# Autodesk Inventor assembly: ChassisFrame-SubAssem01
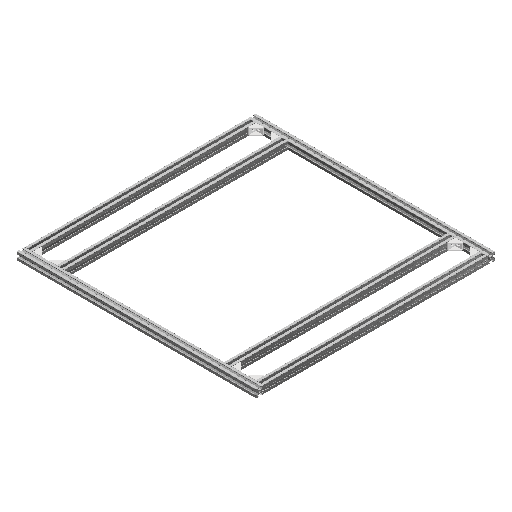
[picture p0: Inventor's stored thumbnail of the model, 512x512]
Saved by Autodesk Inventor 2024 (Build 280153000, 153)
## iProperties
Created: 2022-07-11
Part Number: ChassisFrame-SubAssem01
Document SubType Name: Assembly
Designer: Dave
Author: Dave
## Documents named in this file (5)
- C:\Autodesk\ChalkBot Github\ChalkbotMechanical\Chalkbot1.0\Chassis\V1\ChassisFrame-SubAssem01.iam
- C:\Autodesk\ChalkBot Github\ChalkbotMechanical\Chalkbot1.0\Chassis\V1\20x20 Channel\20x20 Channel-600.ipt
- C:\Users\Dave\Documents\GrabCAD\Chalk Bot\Chalkbot1.0\Chassis\20x20 Channel.ipt
- C:\Autodesk\ChalkBot Github\ChalkbotMechanical\Chalkbot1.0\Chassis\V1\20x20 Channel\20x20 Channel-560.ipt
- C:\Autodesk\ChalkBot Github\ChalkbotMechanical\Chalkbot1.0\Chassis\V1\20x20 90 Gusset.ipt
## Components (14 placed, 3 different names)
1. 20x20 Channel-600:1 — Flush:1, Flush:2, Mate:1, Flush:3, Flush:4, Flush:5, Flush:6, Flush:7, Mate:3, Flush:10, Flush:11, Flush:12, Flush:13, Mate:12, Mate:14, Mate:16, Mate:19
2. 20x20 Channel-600:2 — Flush:1, Flush:2, Mate:2, Mate:4, Mate:7, Mate:8, Mate:10
3. 20x20 Channel-560:3 — Mate:1, Flush:3, Flush:4, Mate:2, Mate:5, Mate:18, Mate:21
4. 20x20 Channel-560:4 — Flush:5, Flush:8, Mate:9, Mate:15, Mate:20
5. 20x20 Channel-560:5 — Flush:7, Flush:9, Mate:3, Flush:10, Flush:14, Flush:15, Flush:16, Flush:17, Flush:18, Mate:11, Mate:13, Mate:20
6. 20x20 Channel-560:6 — Flush:6, Flush:8, Flush:9, Mate:6, Mate:17, Mate:21
7. 20x20 90 Gusset:1 — Flush:11, Mate:12, Mate:13
8. 20x20 90 Gusset:2 — Flush:12, Mate:14, Mate:15
9. 20x20 90 Gusset:3 — Flush:13, Mate:18, Mate:19
10. 20x20 90 Gusset:4 — Flush:14, Mate:16, Mate:17
11. 20x20 90 Gusset:5 — Flush:15, Mate:8, Mate:9
12. 20x20 90 Gusset:6 — Flush:16, Mate:10, Mate:11
13. 20x20 90 Gusset:7 — Flush:17, Mate:6, Mate:7
14. 20x20 90 Gusset:8 — Flush:18, Mate:4, Mate:5
## Relationships (39: Mate 21, Flush 18)
- Flush:1: 20x20 Channel-600:1 ↔ 20x20 Channel-600:2
- Flush:2: 20x20 Channel-600:1 ↔ 20x20 Channel-600:2
- Mate:1: 20x20 Channel-600:1 ↔ 20x20 Channel-560:3
- Flush:3: 20x20 Channel-600:1 ↔ 20x20 Channel-560:3
- Flush:4: 20x20 Channel-600:1 ↔ 20x20 Channel-560:3
- Mate:2: 20x20 Channel-600:2 ↔ 20x20 Channel-560:3
- Flush:5: 20x20 Channel-600:1 ↔ 20x20 Channel-560:4
- Flush:6: 20x20 Channel-600:1 ↔ 20x20 Channel-560:6
- Flush:7: 20x20 Channel-600:1 ↔ 20x20 Channel-560:5
- Flush:8: 20x20 Channel-560:4 ↔ 20x20 Channel-560:6
- Flush:9: 20x20 Channel-560:5 ↔ 20x20 Channel-560:6
- Mate:3: 20x20 Channel-600:1 ↔ 20x20 Channel-560:5
- Flush:10: 20x20 Channel-600:1 ↔ 20x20 Channel-560:5
- Flush:11: 20x20 Channel-600:1 ↔ 20x20 90 Gusset:1
- Flush:12: 20x20 Channel-600:1 ↔ 20x20 90 Gusset:2
- Flush:13: 20x20 Channel-600:1 ↔ 20x20 90 Gusset:3
- Flush:14: 20x20 Channel-560:5 ↔ 20x20 90 Gusset:4
- Flush:15: 20x20 Channel-560:5 ↔ 20x20 90 Gusset:5
- Flush:16: 20x20 Channel-560:5 ↔ 20x20 90 Gusset:6
- Flush:17: 20x20 Channel-560:5 ↔ 20x20 90 Gusset:7
- Flush:18: 20x20 Channel-560:5 ↔ 20x20 90 Gusset:8
- Mate:4: 20x20 Channel-600:2 ↔ 20x20 90 Gusset:8
- Mate:5: 20x20 Channel-560:3 ↔ 20x20 90 Gusset:8
- Mate:6: 20x20 Channel-560:6 ↔ 20x20 90 Gusset:7
- Mate:7: 20x20 Channel-600:2 ↔ 20x20 90 Gusset:7
- Mate:8: 20x20 Channel-600:2 ↔ 20x20 90 Gusset:5
- Mate:9: 20x20 Channel-560:4 ↔ 20x20 90 Gusset:5
- Mate:10: 20x20 Channel-600:2 ↔ 20x20 90 Gusset:6
- Mate:11: 20x20 Channel-560:5 ↔ 20x20 90 Gusset:6
- Mate:12: 20x20 Channel-600:1 ↔ 20x20 90 Gusset:1
- Mate:13: 20x20 Channel-560:5 ↔ 20x20 90 Gusset:1
- Mate:14: 20x20 Channel-600:1 ↔ 20x20 90 Gusset:2
- Mate:15: 20x20 Channel-560:4 ↔ 20x20 90 Gusset:2
- Mate:16: 20x20 Channel-600:1 ↔ 20x20 90 Gusset:4
- Mate:17: 20x20 Channel-560:6 ↔ 20x20 90 Gusset:4
- Mate:18: 20x20 Channel-560:3 ↔ 20x20 90 Gusset:3
- Mate:19: 20x20 Channel-600:1 ↔ 20x20 90 Gusset:3
- Mate:20 (60 mm): 20x20 Channel-560:4 ↔ 20x20 Channel-560:5
- Mate:21 (60 mm): 20x20 Channel-560:3 ↔ 20x20 Channel-560:6
